# Autodesk Inventor assembly: Assembly
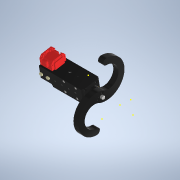
[picture p0: Inventor's stored thumbnail of the model, 180x180]
Saved by Autodesk Inventor 2022 (Build 260153000, 153)
## iProperties
Created: 2022-02-10
Part Number: Assembly
Document SubType Name: Assembly
Designer: br4ch
Author: br4ch
## Documents named in this file (17)
- C:\Users\br4ch\M-and-Ms\HW3\Inventor\Assembly.iam
- C:\Users\br4ch\M-and-Ms\HW3\Inventor\Pipka.ipt
- C:\Users\br4ch\M-and-Ms\HW3\Inventor\Plate.ipt
- C:\Users\br4ch\M-and-Ms\HW3\Inventor\Shaft box.ipt
- C:\Users\br4ch\M-and-Ms\HW3\Inventor\Shaft cap.ipt
- C:\Users\br4ch\M-and-Ms\HW3\Inventor\Shaft.ipt
- C:\Users\br4ch\M-and-Ms\HW3\Inventor\Spacer with a hole.ipt
- C:\Users\br4ch\M-and-Ms\HW3\Inventor\Spacer.ipt
- C:\Users\br4ch\M-and-Ms\HW3\Inventor\Current collector.ipt
- C:\Users\br4ch\M-and-Ms\HW3\Inventor\Disk lapka.ipt
- C:\Users\br4ch\M-and-Ms\HW3\Inventor\Disk.ipt
- C:\Users\br4ch\M-and-Ms\HW3\Inventor\lapka_80_double v3.ipt
- C:\Users\br4ch\M-and-Ms\HW3\Inventor\MX-28T_R v1.ipt
- C:\Users\br4ch\M-and-Ms\HW3\Inventor\bearing.ipt
- C:\Users\br4ch\M-and-Ms\HW3\Inventor\Plate_MIR.ipt
- C:\Users\br4ch\Documents\Inventor\Content Center Files\R2022\en-US\ANSI B18.6.5M(13)\ANSI B18.6.5M - M3x0,5 x 10(32).ipt
- C:\Users\br4ch\Documents\Inventor\Content Center Files\R2022\en-US\ANSI B18.6.5M(09)\ANSI B18.6.5M - M3x0,5 x 10(30).ipt
## Components (27 placed, 16 different names)
1. Pipka:1 — Cylindrical:17, Angle:4, Mate:16
2. Plate:1 — Cylindrical:13, Cylindrical:14, Mate:14, Cylindrical:17, Angle:4, Mate:16, Angle:5, Cylindrical:18, Mate:17
3. Shaft box:1 — Cylindrical:10, Mate:8, Angle:2, Mate:9, Symmetry:1, Mate:10, Mate:11, Symmetry:2, Cylindrical:13, Cylindrical:14, Mate:14, Cylindrical:15, Cylindrical:16, Mate:15
4. Shaft cap:1 — Cylindrical:6, Mate:5, Angle:2, Mate:9, Symmetry:1, Symmetry:2
5. Shaft:1 — Cylindrical:1, Angle:1, Cylindrical:2, Cylindrical:3, Mate:3, Cylindrical:4, Cylindrical:5, Cylindrical:6, Cylindrical:7, Mate:4, Cylindrical:8, Cylindrical:9, Cylindrical:12, Cylindrical:21
6. Spacer with a hole:1 — Mate:12, Cylindrical:12, Mate:13
7. Spacer:1 — Cylindrical:9, Mate:6, Mate:7
8. Current collector:1 — Cylindrical:8, Mate:7, Mate:13
9. Disk lapka:1 — Cylindrical:1, Angle:1, Cylindrical:2, Flush:1, Angle:3, Cylindrical:22, Mate:20
10. Disk:1 — Mate:3, Cylindrical:4, Cylindrical:5, Cylindrical:11
11. lapka_80_double v3:1 — Cylindrical:21, Cylindrical:22, Mate:20
12. MX-28T_R v1:1 — Cylindrical:11, Mate:10, Mate:11
13. Rolling bearing GB/T 7218-1995 Type FSN 70000-Z F 639-Z:1 — Cylindrical:3, Mate:5
14. Rolling bearing GB/T 7218-1995 Type FSN 70000-Z F 639-Z:2 — Cylindrical:7, Mate:4, Mate:6, Cylindrical:10, Mate:8
15. Plate_MIR:1 — Cylindrical:15, Cylindrical:16, Mate:15, Cylindrical:19, Cylindrical:20, Angle:6, Angle:7, Mate:18, Mate:19
16. Pipka:2 — Angle:5, Cylindrical:18, Mate:17
17. Pipka:3 — Cylindrical:19, Angle:6, Mate:18
18. Pipka:4 — Cylindrical:20, Angle:7, Mate:19
19. Cross Recessed Flat Countersunk Head Tapping Screw - Type T - Type IA - Metric M3x0,5 x 10:2
20. Cross Recessed Flat Countersunk Head Tapping Screw - Type D - Type IA - Metric M3x0,5 x 10:1
21. Cross Recessed Flat Countersunk Head Tapping Screw - Type D - Type IA - Metric M3x0,5 x 10:2
22. Cross Recessed Flat Countersunk Head Tapping Screw - Type D - Type IA - Metric M3x0,5 x 10:3
23. Cross Recessed Flat Countersunk Head Tapping Screw - Type D - Type IA - Metric M3x0,5 x 10:4
24. Cross Recessed Flat Countersunk Head Tapping Screw - Type D - Type IA - Metric M3x0,5 x 10:5
25. Cross Recessed Flat Countersunk Head Tapping Screw - Type D - Type IA - Metric M3x0,5 x 10:6
26. Cross Recessed Flat Countersunk Head Tapping Screw - Type D - Type IA - Metric M3x0,5 x 10:7
27. Cross Recessed Flat Countersunk Head Tapping Screw - Type D - Type IA - Metric M3x0,5 x 10:8
## Relationships (58: Mate 26, CylindricalJoint 22, Angle 7, Symmetry 2, Flush 1)
- Cylindrical:1: Shaft:1 ↔ Disk lapka:1
- Angle:1 (0 deg): Shaft:1 ↔ Disk lapka:1
- Cylindrical:2: Shaft:1 ↔ Disk lapka:1
- Flush:1: Disk lapka:1
- Cylindrical:3: Shaft:1 ↔ Rolling bearing GB/T 7218-1995 Type FSN 70000-Z F 639-Z:1
- Mate:3: Shaft:1 ↔ Disk:1
- Cylindrical:4: Shaft:1 ↔ Disk:1
- Cylindrical:5: Shaft:1 ↔ Disk:1
- Cylindrical:6: Shaft cap:1 ↔ Shaft:1
- Cylindrical:7: Shaft:1 ↔ Rolling bearing GB/T 7218-1995 Type FSN 70000-Z F 639-Z:2
- Mate:4: Shaft:1 ↔ Rolling bearing GB/T 7218-1995 Type FSN 70000-Z F 639-Z:2
- Mate:5: Shaft cap:1 ↔ Rolling bearing GB/T 7218-1995 Type FSN 70000-Z F 639-Z:1
- Cylindrical:8: Shaft:1 ↔ Current collector:1
- Cylindrical:9: Shaft:1 ↔ Spacer:1
- Mate:6: Spacer:1 ↔ Rolling bearing GB/T 7218-1995 Type FSN 70000-Z F 639-Z:2
- Mate:7: Spacer:1 ↔ Current collector:1
- Cylindrical:10: Shaft box:1 ↔ Rolling bearing GB/T 7218-1995 Type FSN 70000-Z F 639-Z:2
- Mate:8: Shaft box:1 ↔ Rolling bearing GB/T 7218-1995 Type FSN 70000-Z F 639-Z:2
- Angle:2 (0 deg): Shaft box:1 ↔ Shaft cap:1
- Mate:9: Shaft box:1 ↔ Shaft cap:1
- Symmetry:1: Shaft box:1 ↔ Shaft cap:1
- Angle:3 (0 deg): Disk lapka:1
- Cylindrical:11: Disk:1 ↔ MX-28T_R v1:1
- Mate:10: Shaft box:1 ↔ MX-28T_R v1:1
- Mate:11: Shaft box:1 ↔ MX-28T_R v1:1
- Symmetry:2: Shaft box:1 ↔ Shaft cap:1
- Mate:12: Spacer with a hole:1
- Cylindrical:12: Shaft:1 ↔ Spacer with a hole:1
- Mate:13: Spacer with a hole:1 ↔ Current collector:1
- Cylindrical:13: Plate:1 ↔ Shaft box:1
- Cylindrical:14: Plate:1 ↔ Shaft box:1
- Mate:14: Plate:1 ↔ Shaft box:1
- Cylindrical:15: Shaft box:1 ↔ Plate_MIR:1
- Cylindrical:16: Shaft box:1 ↔ Plate_MIR:1
- Mate:15: Shaft box:1 ↔ Plate_MIR:1
- Cylindrical:17: Pipka:1 ↔ Plate:1
- Angle:4 (0 deg): Pipka:1 ↔ Plate:1
- Mate:16: Pipka:1 ↔ Plate:1
- Angle:5 (0 deg): Plate:1 ↔ Pipka:2
- Cylindrical:18: Plate:1 ↔ Pipka:2
- Mate:17: Plate:1 ↔ Pipka:2
- Cylindrical:19: Plate_MIR:1 ↔ Pipka:3
- Cylindrical:20: Plate_MIR:1 ↔ Pipka:4
- Angle:6 (0 deg): Plate_MIR:1 ↔ Pipka:3
- Angle:7 (0 deg): Plate_MIR:1 ↔ Pipka:4
- Mate:18: Plate_MIR:1 ↔ Pipka:3
- Mate:19: Plate_MIR:1 ↔ Pipka:4
- Cylindrical:21: Shaft:1 ↔ lapka_80_double v3:1
- Cylindrical:22: Disk lapka:1 ↔ lapka_80_double v3:1
- Mate:20: Disk lapka:1 ↔ lapka_80_double v3:1
- [Mate]: Plate_MIR:1 ↔ Cross Recessed Flat Countersunk Head Tapping Screw - Type D - Type IA - Metric M3x0,5 x 10:1
- [Mate]: Plate_MIR:1 ↔ Cross Recessed Flat Countersunk Head Tapping Screw - Type D - Type IA - Metric M3x0,5 x 10:2
- [Mate]: Plate_MIR:1 ↔ Cross Recessed Flat Countersunk Head Tapping Screw - Type D - Type IA - Metric M3x0,5 x 10:3
- [Mate]: Plate_MIR:1 ↔ Cross Recessed Flat Countersunk Head Tapping Screw - Type D - Type IA - Metric M3x0,5 x 10:4
- [Mate]: Plate:1 ↔ Cross Recessed Flat Countersunk Head Tapping Screw - Type D - Type IA - Metric M3x0,5 x 10:5
- [Mate]: Plate:1 ↔ Cross Recessed Flat Countersunk Head Tapping Screw - Type D - Type IA - Metric M3x0,5 x 10:6
- [Mate]: Plate:1 ↔ Cross Recessed Flat Countersunk Head Tapping Screw - Type D - Type IA - Metric M3x0,5 x 10:7
- [Mate]: Plate:1 ↔ Cross Recessed Flat Countersunk Head Tapping Screw - Type D - Type IA - Metric M3x0,5 x 10:8
